# Autodesk Inventor assembly: Stamp Assembly
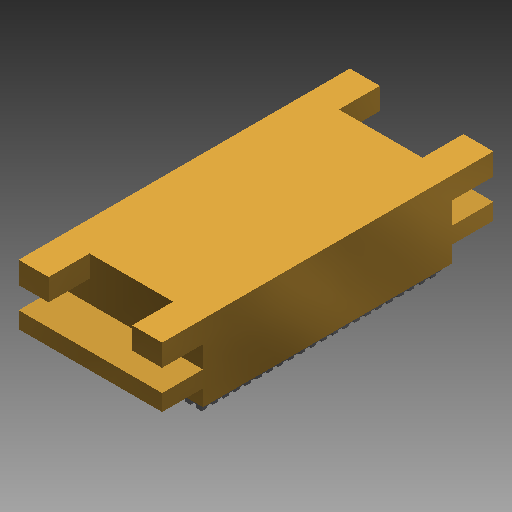
[picture p0: Inventor's stored thumbnail of the model, 512x512]
Saved by Autodesk Inventor 2019.4 (Build 234330000, 330)
## iProperties
Created: 2021-01-06
Part Number: Stamp Assembly
Document SubType Name: Assembly
Designer: caleb
Author: caleb
## Documents named in this file (3)
- C:\Users\cfang\Desktop\nebraska-silicon-lab\Hardware\ETL\Module Assembly\Glue Stamp\Stamp Assembly.iam
- C:\Users\cfang\Desktop\nebraska-silicon-lab\Hardware\ETL\Module Assembly\Glue Stamp\Rubber Stamp.ipt
- C:\Users\cfang\Desktop\nebraska-silicon-lab\Hardware\ETL\Module Assembly\Glue Stamp\Stamp Body.ipt
## Components (2 placed, 2 different names)
1. Rubber Stamp:1 — Mate:1
2. Stamp Body:1 — Mate:1
## Relationships (1: Mate 1)
- Mate:1: Rubber Stamp:1 ↔ Stamp Body:1
